# Autodesk Inventor assembly: ASY PNS 1710 charging hatch
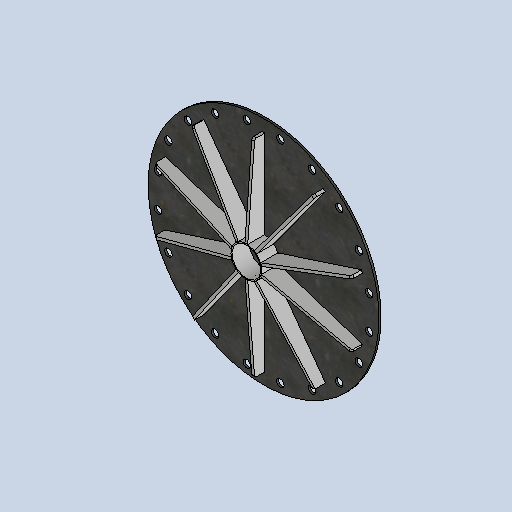
[picture p0: Inventor's stored thumbnail of the model, 512x512]
Saved by Autodesk Inventor 2025.1 (Build 291241020, 241B)
## iProperties
Created: 2025-04-22
Part Number: ASY PNS 1710 charging hatch
Document SubType Name: Assembly
Designer: user
Author: user
## Documents named in this file (4)
- C:\Users\user\YandexDisk-badmisterfox\home pc\Inventor\PNS2-Panaevsk\Filter D1000\ASY PNS 1710 charging hatch.iam
- C:\Users\user\YandexDisk-badmisterfox\home pc\Inventor\PNS2-Panaevsk\Filter D1200\PNS 1712 charging hatch 500mm.ipt
- C:\Users\user\YandexDisk-badmisterfox\home pc\Inventor\PNS2-Panaevsk\Filter D1200\PNS 1713 charging hatch reinf 500mm.ipt
- C:\Users\user\YandexDisk-badmisterfox\home pc\Inventor\PNS2-Panaevsk\Filter D1200\PNS 1711 hatch tube 500mm.ipt
## Components (12 placed, 3 different names)
1. PNS 1712 charging hatch 500mm.ipt:1 — Rigid:1, Flush:1
2. PNS 1711 hatch tube 500mm.ipt:1 — Rigid:1
3. PNS 1713 charging hatch reinf 500mm.ipt:1 — Mate:1, Flush:1, Mate:2, Mate:3
4. PNS 1713 charging hatch reinf 500mm.ipt:2
5. PNS 1713 charging hatch reinf 500mm.ipt:3
6. PNS 1713 charging hatch reinf 500mm.ipt:4
7. PNS 1713 charging hatch reinf 500mm.ipt:5
8. PNS 1713 charging hatch reinf 500mm.ipt:6
9. PNS 1713 charging hatch reinf 500mm.ipt:7
10. PNS 1713 charging hatch reinf 500mm.ipt:8
11. PNS 1713 charging hatch reinf 500mm.ipt:9
12. PNS 1713 charging hatch reinf 500mm.ipt:10
## Component patterns: (10 elements, first: PNS 1713 charging hatch reinf 500mm.ipt:1)
## Relationships (5: Mate 3, WeldJoint 1, Flush 1)
- Rigid:1 [WeldJoint]: PNS 1712 charging hatch 500mm.ipt:1 ↔ PNS 1711 hatch tube 500mm.ipt:1
- Mate:1: PNS 1713 charging hatch reinf 500mm.ipt:1
- Flush:1: PNS 1712 charging hatch 500mm.ipt:1 ↔ PNS 1713 charging hatch reinf 500mm.ipt:1
- Mate:2: PNS 1713 charging hatch reinf 500mm.ipt:1
- Mate:3: PNS 1713 charging hatch reinf 500mm.ipt:1
